# Autodesk Inventor assembly: drive-train
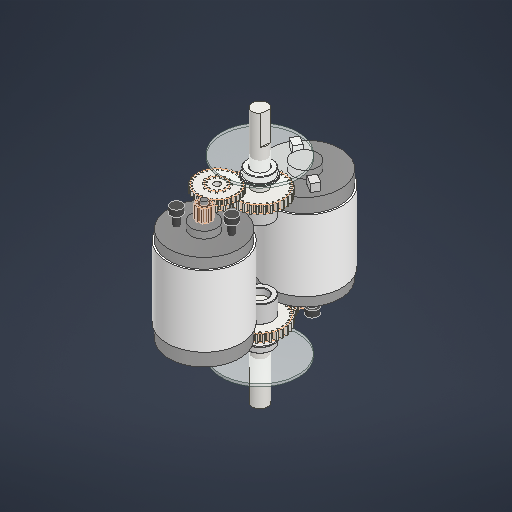
[picture p0: Inventor's stored thumbnail of the model, 512x512]
Saved by Autodesk Inventor 2026.2 (Build 302298000, 298)
## iProperties
Created: 2026-03-09
Part Number: drive-train
Document SubType Name: Assembly
Designer: szymo
Author: szymo
## Documents named in this file (9)
- C:\Users\szymo\Downloads\evangelion-turbo\inventor-project\drive-train.iam
- C:\Users\szymo\Downloads\evangelion-turbo\inventor-project\rs385.ipt
- C:\Users\szymo\Downloads\evangelion-turbo\inventor-project\gear-smol.iam
- C:\Users\szymo\Downloads\evangelion-turbo\inventor-project\gear-stack-big.iam
- C:\Users\szymo\Downloads\evangelion-turbo\inventor-project\oska-assembly.iam
- C:\Users\szymo\Downloads\evangelion-turbo\inventor-project\kolo-atrapa.ipt
- C:\Users\szymo\Downloads\evangelion-turbo\inventor-project\metal_shield.ipt
- C:\Users\szymo\Downloads\evangelion-turbo\inventor-project\screw_for_motors.ipt
- C:\Users\szymo\Downloads\evangelion-turbo\inventor-project\TFMINI_S_UART.ipt
## Components (16 placed, 7 different names)
1. rs385:1 — Tangent:1, Tangent:2, Flush:1, Angle:1, Mate:3, Tangent:6, Mate:5, Mate:6, Mate:18, Tangent:11, Tangent:13, Tangent:16, Mate:19, Flush:5, Flush:9, Flush:10, Mate:23, Mate:24, Angle:2
2. rs385:2 — Tangent:3, Angle:1, Tangent:6, Mate:9, Mate:10, Mate:11, Tangent:12, Tangent:14, Tangent:15, Mate:20, Flush:6, Flush:7, Flush:8, Mate:21, Mate:22, Angle:3
3. gear-smol:1 [sub-assembly] — Mate:3, Tangent:4, Mate:6
4. gear-stack-big:1 [sub-assembly] — Tangent:4, Tangent:5, Mate:5, Flush:2, Tangent:16
5. oska-assembly:1 [sub-assembly] — Mate:1, Mate:2, Tangent:5, Flush:2, Mate:12, Tangent:13, Tangent:14
6. kolo-atrapa:1 — Mate:1, Mate:2, Tangent:7
7. gear-smol:2 [sub-assembly] — Mate:9, Mate:10, Tangent:8
8. gear-stack-big:2 [sub-assembly] — Mate:11, Flush:4, Tangent:8, Tangent:9, Tangent:15
9. oska-assembly:2 [sub-assembly] — Flush:4, Tangent:9, Mate:12, Mate:18, Tangent:11, Tangent:12
10. kolo-atrapa:2 — Tangent:10
11. metal_shield:1 — Mate:19, Flush:5
12. metal_shield:2 — Mate:20, Flush:6
13. screw_for_motors:1 — Flush:10, Mate:24
14. screw_for_motors:2 — Flush:7, Mate:21
15. screw_for_motors:3 — Flush:9, Mate:23
16. screw_for_motors:4 — Flush:8, Mate:22
## Relationships (46: Mate 18, Tangent 16, Flush 9, Angle 3)
- Tangent:1: rs385:1
- Tangent:2: rs385:1
- Flush:1: rs385:1
- Tangent:3: rs385:2
- Angle:1 (180 deg): rs385:1 ↔ rs385:2
- Mate:1: oska-assembly:1 ↔ kolo-atrapa:1
- Mate:2 (10 mm): oska-assembly:1 ↔ kolo-atrapa:1
- Mate:3: rs385:1 ↔ gear-smol:1
- Tangent:4: gear-smol:1 ↔ gear-stack-big:1
- Tangent:5: gear-stack-big:1 ↔ oska-assembly:1
- Tangent:6 (16 mm): rs385:1 ↔ rs385:2
- Tangent:7 (-2.65 mm): kolo-atrapa:1
- Mate:5 (2 mm): rs385:1 ↔ gear-stack-big:1
- Mate:6 (1 mm): rs385:1 ↔ gear-smol:1
- Flush:2: gear-stack-big:1 ↔ oska-assembly:1
- [Mate]: oska-assembly:2 ↔ kolo-atrapa:2
- [Mate] (10 mm): oska-assembly:2 ↔ kolo-atrapa:2
- Mate:9: rs385:2 ↔ gear-smol:2
- Mate:10 (1 mm): rs385:2 ↔ gear-smol:2
- Mate:11 (2 mm): rs385:2 ↔ gear-stack-big:2
- Flush:4: gear-stack-big:2 ↔ oska-assembly:2
- Tangent:8: gear-smol:2 ↔ gear-stack-big:2
- Tangent:9: gear-stack-big:2 ↔ oska-assembly:2
- Tangent:10 (-2.65 mm): kolo-atrapa:2
- Mate:12: oska-assembly:1 ↔ oska-assembly:2
- Mate:18 (1.4 mm): rs385:1 ↔ oska-assembly:2
- Tangent:11 (1.665 mm): rs385:1 ↔ oska-assembly:2
- Tangent:12 (0.5 mm): rs385:2 ↔ oska-assembly:2
- Tangent:13 (1.665 mm): rs385:1 ↔ oska-assembly:1
- Tangent:14 (0.5 mm): rs385:2 ↔ oska-assembly:1
- Tangent:15 (3.75 mm): rs385:2 ↔ gear-stack-big:2
- Tangent:16 (3.75 mm): rs385:1 ↔ gear-stack-big:1
- Mate:19: rs385:1 ↔ metal_shield:1
- Mate:20: rs385:2 ↔ metal_shield:2
- Flush:5 (-4 mm): rs385:1 ↔ metal_shield:1
- Flush:6 (4 mm): rs385:2 ↔ metal_shield:2
- Flush:7 (-6.5 mm): rs385:2 ↔ screw_for_motors:2
- Flush:8 (6.5 mm): rs385:2 ↔ screw_for_motors:4
- Mate:21: rs385:2 ↔ screw_for_motors:2
- Mate:22: rs385:2 ↔ screw_for_motors:4
- Flush:9 (-6.5 mm): rs385:1 ↔ screw_for_motors:3
- Flush:10 (-6.5 mm): rs385:1 ↔ screw_for_motors:1
- Mate:23: rs385:1 ↔ screw_for_motors:3
- Mate:24: rs385:1 ↔ screw_for_motors:1
- Angle:2 (-60 deg): rs385:1
- Angle:3 (-60 deg): rs385:2
## Named parameters: d22_d6 = 0 mm, d23_d7 = 10 mm
